# Autodesk Inventor assembly: Assembly1
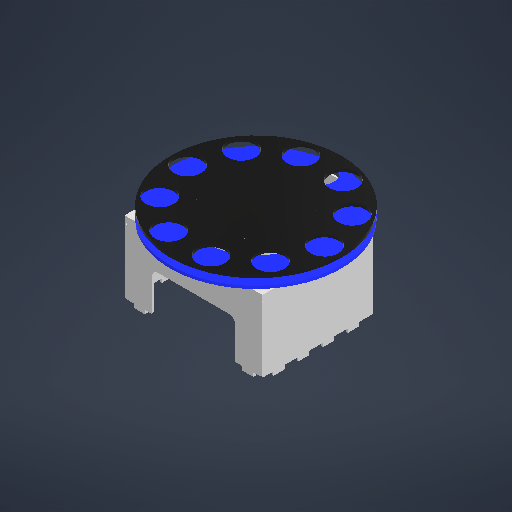
[picture p0: Inventor's stored thumbnail of the model, 512x512]
Saved by Autodesk Inventor 2027.1 (Build 311270010, 270A)
## iProperties
Created: 2026-09-28
Part Number: Assembly1
Document SubType Name: Assembly
Designer: daniel
Author: daniel
## Documents named in this file (10)
- C:\Users\danda\Documents\GitHub\MCT333_Design_of_Mechatronics_Systems_1\CAD\FEED and Sorting\Assembly1.iam
- C:\Users\danda\Documents\GitHub\MCT333_Design_of_Mechatronics_Systems_1\CAD\FEED and Sorting\Part2.ipt
- C:\Users\danda\Documents\GitHub\MCT333_Design_of_Mechatronics_Systems_1\CAD\FEED and Sorting\Part1.ipt
- C:\Users\danda\Documents\GitHub\MCT333_Design_of_Mechatronics_Systems_1\CAD\off_the_shelf_components\standard-servo-motor-black-1.snapshot.7\Assem1\Assem1.iam
- C:\Users\danda\Documents\GitHub\MCT333_Design_of_Mechatronics_Systems_1\CAD\FEED and Sorting\Part22.ipt
- C:\Users\danda\Documents\GitHub\MCT333_Design_of_Mechatronics_Systems_1\CAD\FEED and Sorting\Part27.ipt
- C:\Users\danda\Documents\GitHub\MCT333_Design_of_Mechatronics_Systems_1\CAD\FEED and Sorting\Part67.ipt
- C:\Users\danda\Documents\Inventor\Content Center Files\R2027\en-US\GB_T 301-1995(51000)\Rolling bearing 51109 GB_T 301-1995.ipt
- C:\Users\danda\Documents\GitHub\MCT333_Design_of_Mechatronics_Systems_1\CAD\FEED and Sorting\Part69.ipt
- C:\Users\danda\Documents\GitHub\MCT333_Design_of_Mechatronics_Systems_1\CAD\FEED and Sorting\box\MagazineBox.iam
## Components (10 placed, 9 different names)
1. Part2:1 — Mate:13, Mate:14, Mate:15, Mate:16
2. Part1:1 — Mate:2, Mate:3, Mate:5, Mate:6, Mate:7, Mate:8, Mate:12, Mate:18, Mate:20
3. Assem1:1 [sub-assembly] — Mate:9, Mate:10, Mate:11, Mate:16
4. Part22:1 — Tangent:3, Mate:20
5. Part27:1 — Mate:18, Tangent:3
6. Part67:1 — Mate:4, Flush:2, Mate:5, Flush:3
7. Rolling bearing GB/T 301-1995 Type 51000 51109:1 — Mate:12, Tangent:1, Tangent:2
8. Part69:1 — Mate:13, Mate:14, Mate:15, Tangent:2
9. Part69:2 — Mate:6, Mate:7, Mate:8, Tangent:1
10. MagazineBox:1 [sub-assembly] — Mate:2, Mate:3, Mate:4, Flush:2, Mate:9, Mate:10, Mate:11, Flush:3
## Relationships (22: Mate 17, Tangent 3, Flush 2)
- Mate:2: Part1:1 ↔ MagazineBox:1
- Mate:3: Part1:1 ↔ MagazineBox:1
- Mate:4: Part67:1 ↔ MagazineBox:1
- Flush:2: Part67:1 ↔ MagazineBox:1
- Mate:5: Part1:1 ↔ Part67:1
- Mate:6: Part1:1 ↔ Part69:2
- Mate:7: Part1:1 ↔ Part69:2
- Mate:8: Part1:1 ↔ Part69:2
- Mate:9: Assem1:1 ↔ MagazineBox:1
- Mate:10: Assem1:1 ↔ MagazineBox:1
- Mate:11: Assem1:1 ↔ MagazineBox:1
- Mate:12: Part1:1 ↔ Rolling bearing GB/T 301-1995 Type 51000 51109:1
- Tangent:1: Rolling bearing GB/T 301-1995 Type 51000 51109:1 ↔ Part69:2
- Mate:13: Part2:1 ↔ Part69:1
- Mate:14: Part2:1 ↔ Part69:1
- Mate:15: Part2:1 ↔ Part69:1
- Tangent:2: Rolling bearing GB/T 301-1995 Type 51000 51109:1 ↔ Part69:1
- Mate:16: Part2:1 ↔ Assem1:1
- Mate:18: Part1:1 ↔ Part27:1
- Tangent:3: Part22:1 ↔ Part27:1
- Mate:20: Part1:1 ↔ Part22:1
- Flush:3: Part67:1 ↔ MagazineBox:1
